# Autodesk Inventor assembly: obj1
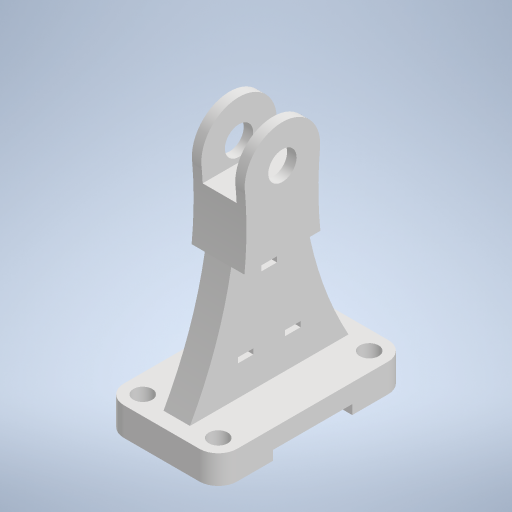
[picture p0: Inventor's stored thumbnail of the model, 512x512]
Saved by Autodesk Inventor 2023.2 (Build 272271030, 271C)
## iProperties
Created: 2023-02-25
Part Number: obj1
Document SubType Name: Assembly
Designer: Cris Pat
Author: Cris Pat
## Documents named in this file (7)
- C:\Users\Cris Pat\Desktop\U\Semestre 9\disenio e innovacion\CAD\obj1.iam
- C:\Users\Cris Pat\Documents\Inventor\Content Center Files\R2023\en-US\DIN 84\DIN 84 - M5 x 20.ipt
- C:\Users\Cris Pat\Documents\Inventor\Content Center Files\R2023\en-US\DIN 439-2\DIN 439 - M5 x 0.8.ipt
- C:\Users\Cris Pat\Desktop\U\Semestre 9\disenio e innovacion\CAD\base_obj1.ipt
- C:\Users\Cris Pat\Desktop\U\Semestre 9\disenio e innovacion\CAD\cuerpo_obj1.ipt
- C:\Users\Cris Pat\Documents\Inventor\Content Center Files\R2023\en-US\DIN 84\DIN 84 - M5 x 30.ipt
- C:\Users\Cris Pat\Desktop\U\Semestre 9\disenio e innovacion\CAD\cabeza_obj1.ipt
## Components (9 placed, 6 different names)
1. DIN 84 - replaced by DIN EN ISO 1207 M5 x 20:1 — Rotational:5
2. base_obj1:1 — Rigid:1, Rigid:2, Rigid:3
3. cuerpo_obj1:1 — Rigid:1, Rotational:2, Rotational:3, Rotational:4, Rigid:4
4. DIN 84 - replaced by DIN EN ISO 1207 M5 x 30:1 — Rigid:2
5. DIN 84 - replaced by DIN EN ISO 1207 M5 x 30:2 — Rigid:3
6. DIN 439-2 - replaced by DIN EN 24035/28675 M5:2 — Rotational:2
7. DIN 439-2 - replaced by DIN EN 24035/28675 M5:3 — Rotational:4
8. DIN 439-2 - replaced by DIN EN 24035/28675 M5:4 — Rotational:3
9. cabeza_obj1:1 — Rotational:5, Rigid:4
## Relationships (8: WeldJoint 4, RevoluteJoint 4)
- Rigid:1 [WeldJoint]: base_obj1:1 ↔ cuerpo_obj1:1
- Rigid:2 [WeldJoint]: base_obj1:1 ↔ DIN 84 - replaced by DIN EN ISO 1207 M5 x 30:1
- Rotational:2 [RevoluteJoint]: cuerpo_obj1:1 ↔ DIN 439-2 - replaced by DIN EN 24035/28675 M5:2
- Rotational:3 [RevoluteJoint]: cuerpo_obj1:1 ↔ DIN 439-2 - replaced by DIN EN 24035/28675 M5:4
- Rigid:3 [WeldJoint]: base_obj1:1 ↔ DIN 84 - replaced by DIN EN ISO 1207 M5 x 30:2
- Rotational:4 [RevoluteJoint]: cuerpo_obj1:1 ↔ DIN 439-2 - replaced by DIN EN 24035/28675 M5:3
- Rotational:5 [RevoluteJoint]: DIN 84 - replaced by DIN EN ISO 1207 M5 x 20:1 ↔ cabeza_obj1:1
- Rigid:4 [WeldJoint]: cuerpo_obj1:1 ↔ cabeza_obj1:1
